# Autodesk Inventor assembly: InsertAssembly
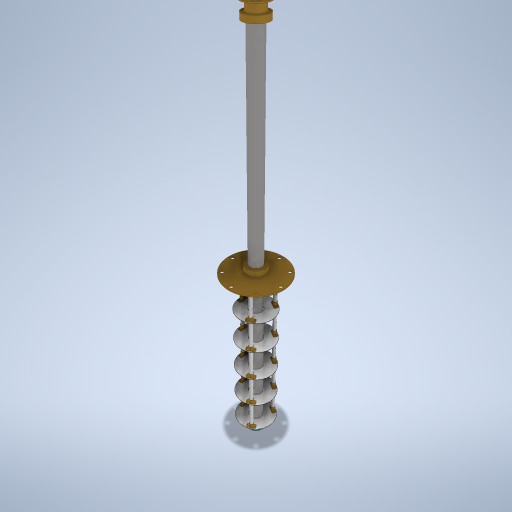
[picture p0: Inventor's stored thumbnail of the model, 512x512]
Saved by Autodesk Inventor 2024 (Build 280153000, 153)
## iProperties
Created: 2023-11-04
Part Number: InsertAssembly
Document SubType Name: Assembly
Designer: schanen
Author: schanen
## Documents named in this file (3)
- C:\Users\schanen\Documents\Inventor\LargeTransportDewarInsert2023\pdfs\InsertAssembly.iam
- C:\Users\schanen\Documents\Inventor\LargeTransportDewarInsert2023\Insert.iam
- C:\Users\schanen\Documents\Inventor\LargeTransportDewarInsert2023\SlidingAssembly.iam
## Components (2 placed, 2 different names)
1. Insert:1 [sub-assembly]
2. SlidingAssembly:1 [sub-assembly]
## Relationships (1: Mate 1)
- [Mate]: Insert:1 ↔ SlidingAssembly:1
